# Autodesk Inventor assembly: BREEZE-S06
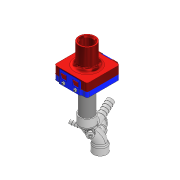
[picture p0: Inventor's stored thumbnail of the model, 180x180]
Saved by Autodesk Inventor 2020 (Build 240168000, 168)
## iProperties
Created: 2020-04-12
Part Number: BREEZE-S06
Document SubType Name: Assembly
Designer: John K
Description: OUTLET ASSEMBLY
Author: John K
## Documents named in this file (14)
- C:\GrabCAD\MTL Ventilator Design\BREEZE\Subassemblies\BREEZE-S06.iam
- C:\GrabCAD\MTL Ventilator Design\BREEZE\Manufactured Parts\BREEZE-M24.ipt
- C:\GrabCAD\MTL Ventilator Design\BREEZE\Manufactured Parts\BREEZE-M13.ipt
- C:\GrabCAD\MTL Ventilator Design\BREEZE\Commercial Parts\McMaster\M3 Insert.ipt
- C:\GrabCAD\MTL Ventilator Design\BREEZE\Commercial Parts\Electronics\Flow Sensor.ipt
- C:\GrabCAD\MTL Ventilator Design\BREEZE\Manufactured Parts\BREEZE-M21.ipt
- C:\GrabCAD\MTL Ventilator Design\BREEZE\Commercial Parts\McMaster\M3x8mm Socket.ipt
- C:\GrabCAD\MTL Ventilator Design\BREEZE\Commercial Parts\McMaster\M3x6mm Nylon Screw.ipt
- C:\GrabCAD\MTL Ventilator Design\BREEZE\Commercial Parts\McMaster\M4x35mm Nylon Screw.ipt
- C:\GrabCAD\MTL Ventilator Design\BREEZE\Commercial Parts\McMaster\Pressure Relief Vent.ipt
- C:\GrabCAD\MTL Ventilator Design\BREEZE\Commercial Parts\McMaster\Oxygen Sensor.ipt
- C:\GrabCAD\MTL Ventilator Design\BREEZE\Manufactured Parts\BREEZE-M22.ipt
- C:\GrabCAD\MTL Ventilator Design\BREEZE\Manufactured Parts\BREEZE-M25.ipt
- C:\GrabCAD\MTL Ventilator Design\BREEZE\Commercial Parts\McMaster\O-Ring Dash 036 Square.ipt
## Components (19 placed, 13 different names)
1. BREEZE-M13:1 — Insert:15, Insert:20
2. BREEZE-M21:1 — Insert:6, Angle:2, Insert:22, Insert:23
3. BREEZE-M22:1 — Mate:1, Flush:1, Mate:7, Mate:2, Flush:3, Angle:1, Mate:3, Flush:4, Insert:4, Insert:8, Insert:9, Insert:10, Insert:11, Insert:15, Insert:17, Mate:8, Insert:3, Mate:9, Mate:10, Mate:11
4. BREEZE-M24:1 — Mate:2, Flush:3, Angle:1, Insert:21
5. BREEZE-M25:1 — Mate:3, Flush:4, Insert:18, Insert:19, Mate:8
6. Flow Sensor:1 — Insert:6, Insert:17
7. Oxygen Sensor:1 — Insert:23
8. Pressure Relief Vent:1 — Insert:22
9. O-Ring Dash 036 Square:1 — Mate:9, Mate:10, Mate:11
10. M4x35mm Nylon Screw:1 — Insert:21
11. M3x8mm Socket:2 — Insert:8
12. M3x8mm Socket:3 — Insert:9
13. M3x8mm Socket:4 — Insert:10
14. M3x8mm Socket:5 — Insert:11
15. M3x6mm Nylon Screw:1 — Insert:18
16. M3x6mm Nylon Screw:2 — Insert:19
17. M3x6mm Nylon Screw:3 — Insert:20
18. M3 Insert:1 — Insert:3
19. M3 Insert:2 — Insert:4
## Relationships (28: Insert 15, Mate 8, Flush 3, Angle 2)
- Mate:1: BREEZE-M22:1
- Flush:1: BREEZE-M22:1
- Mate:7: BREEZE-M22:1
- Mate:2: BREEZE-M22:1 ↔ BREEZE-M24:1
- Flush:3: BREEZE-M22:1 ↔ BREEZE-M24:1
- Angle:1 (180 deg): BREEZE-M22:1 ↔ BREEZE-M24:1
- Mate:3: BREEZE-M22:1 ↔ BREEZE-M25:1
- Flush:4: BREEZE-M22:1 ↔ BREEZE-M25:1
- Insert:3: BREEZE-M22:1 ↔ M3 Insert:1
- Insert:4: BREEZE-M22:1 ↔ M3 Insert:2
- Insert:6: BREEZE-M21:1 ↔ Flow Sensor:1
- Angle:2 (42 deg): BREEZE-M21:1
- Insert:8: BREEZE-M22:1 ↔ M3x8mm Socket:2
- Insert:9: BREEZE-M22:1 ↔ M3x8mm Socket:3
- Insert:10: BREEZE-M22:1 ↔ M3x8mm Socket:4
- Insert:11: BREEZE-M22:1 ↔ M3x8mm Socket:5
- Insert:15: BREEZE-M13:1 ↔ BREEZE-M22:1
- Insert:17: BREEZE-M22:1 ↔ Flow Sensor:1
- Insert:18: BREEZE-M25:1 ↔ M3x6mm Nylon Screw:1
- Insert:19: BREEZE-M25:1 ↔ M3x6mm Nylon Screw:2
- Insert:20: BREEZE-M13:1 ↔ M3x6mm Nylon Screw:3
- Insert:21: BREEZE-M24:1 ↔ M4x35mm Nylon Screw:1
- Insert:22: BREEZE-M21:1 ↔ Pressure Relief Vent:1
- Insert:23: BREEZE-M21:1 ↔ Oxygen Sensor:1
- Mate:8: BREEZE-M22:1 ↔ BREEZE-M25:1
- Mate:9: BREEZE-M22:1 ↔ O-Ring Dash 036 Square:1
- Mate:10: BREEZE-M22:1 ↔ O-Ring Dash 036 Square:1
- Mate:11: BREEZE-M22:1 ↔ O-Ring Dash 036 Square:1
